# Autodesk Inventor assembly: Solenoid
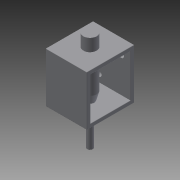
[picture p0: Inventor's stored thumbnail of the model, 180x180]
Saved by Autodesk Inventor 2015 (Build 190159000, 159)
## iProperties
Created: 2015-11-10
Part Number: Solenoid
Document SubType Name: Assembly
Designer: Lauszus
Author: Lauszus
## Documents named in this file (3)
- C:\Users\Lauszus\Dropbox\DTU\7. semester\Image Analysis with Microcomputer - 30330\Lab exercises\ObjectTracking\3DModel\Solenoid.iam
- C:\Users\Lauszus\Dropbox\DTU\7. semester\Image Analysis with Microcomputer - 30330\Lab exercises\ObjectTracking\3DModel\Solenoid_shell.ipt
- C:\Users\Lauszus\Dropbox\DTU\7. semester\Image Analysis with Microcomputer - 30330\Lab exercises\ObjectTracking\3DModel\Solenoid_pin.ipt
## Components (2 placed, 2 different names)
1. Solenoid_shell:1 — Mate:1, Mate:2
2. Solenoid_pin:1 — Mate:1, Mate:2
## Relationships (2: Mate 2)
- Mate:1: Solenoid_shell:1 ↔ Solenoid_pin:1
- Mate:2: Solenoid_shell:1 ↔ Solenoid_pin:1
